# Autodesk Inventor assembly: Stowed CubSat Assembly
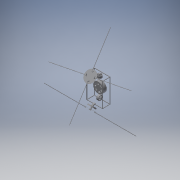
[picture p0: Inventor's stored thumbnail of the model, 180x180]
Saved by Autodesk Inventor 2016 (Build 200138000, 138)
## iProperties
Created: 2015-12-21
Part Number: Stowed CubSat Assembly
Document SubType Name: Assembly
Designer: jonathan
Author: jonathan
## Documents named in this file (8)
- C:\Users\jonathan\Dropbox\Satellite\CAD\Locked CubeSat Assembly.iam
- C:\Users\jonathan\Dropbox\Satellite\CAD\CubeSat Frame.ipt
- C:\Users\jonathan\Dropbox\Satellite\CAD\Spinning Platform.ipt
- C:\Users\jonathan\Dropbox\Satellite\CAD\Motor Assembly.iam
- C:\Users\jonathan\Dropbox\Satellite\CAD\Large Flywheel.ipt
- C:\Users\jonathan\Dropbox\Satellite\CAD\Orthogonal Bracket.ipt
- C:\Users\jonathan\Dropbox\Satellite\CAD\Flywheel Bracket.ipt
- C:\Users\jonathan\Dropbox\Satellite\CAD\Small Flywheel.ipt
## Components (13 placed, 7 different names)
1. CubeSat Frame:1 — Mate:4, Flush:3, Mate:6, Flush:4, Flush:5, Flush:6, Flush:7
2. Motor Assembly:1 [sub-assembly] — Mate:5, Rigid:1, Mate:7, Mate:8
3. Motor Assembly:2 [sub-assembly] — Rigid:2, Mate:9, Insert:1
4. Large Flywheel:1 — Mate:10, Insert:2
5. Orthogonal Bracket:1 — Mate:4, Flush:3, Mate:5, Rigid:1
6. Orthogonal Bracket:2 — Mate:6, Flush:4, Rigid:2
7. Spinning Platform:1 — Mate:7, Mate:8
8. Spinning Platform:2 — Mate:9, Insert:1
9. Flywheel Bracket:1 — Flush:6, Mate:12, Mate:13
10. Flywheel Bracket:2 — Flush:5, Mate:10, Insert:2
11. Flywheel Bracket:3 — Flush:7, Mate:11, Insert:3
12. Small Flywheel:1 — Mate:11, Insert:3
13. Small Flywheel:2 — Mate:12, Mate:13
## Relationships (20: Mate 10, Flush 5, Insert 3, WeldJoint 2)
- Mate:4: CubeSat Frame:1 ↔ Orthogonal Bracket:1
- Flush:3: CubeSat Frame:1 ↔ Orthogonal Bracket:1
- Mate:5: Motor Assembly:1 ↔ Orthogonal Bracket:1
- Rigid:1 [WeldJoint]: Motor Assembly:1 ↔ Orthogonal Bracket:1
- Mate:6: CubeSat Frame:1 ↔ Orthogonal Bracket:2
- Flush:4: CubeSat Frame:1 ↔ Orthogonal Bracket:2
- Rigid:2 [WeldJoint]: Motor Assembly:2 ↔ Orthogonal Bracket:2
- Mate:7: Motor Assembly:1 ↔ Spinning Platform:1
- Mate:8: Motor Assembly:1 ↔ Spinning Platform:1
- Mate:9: Motor Assembly:2 ↔ Spinning Platform:2
- Insert:1: Motor Assembly:2 ↔ Spinning Platform:2
- Flush:5: CubeSat Frame:1 ↔ Flywheel Bracket:2
- Mate:10: Large Flywheel:1 ↔ Flywheel Bracket:2
- Insert:2: Large Flywheel:1 ↔ Flywheel Bracket:2
- Flush:6: CubeSat Frame:1 ↔ Flywheel Bracket:1
- Flush:7 (76.2 mm): CubeSat Frame:1 ↔ Flywheel Bracket:3
- Mate:11: Flywheel Bracket:3 ↔ Small Flywheel:1
- Insert:3: Flywheel Bracket:3 ↔ Small Flywheel:1
- Mate:12: Flywheel Bracket:1 ↔ Small Flywheel:2
- Mate:13: Flywheel Bracket:1 ↔ Small Flywheel:2
